# Autodesk Inventor assembly: Diamond-Box-Assembly
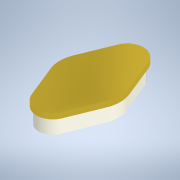
[picture p0: Inventor's stored thumbnail of the model, 180x180]
Saved by Autodesk Inventor 2022.4 (Build 264492000, 492)
## iProperties
Created: 2024-03-07
Part Number: Diamond-Box-Assembly
Document SubType Name: Assembly
Designer: t60147996
Author: t60147996
## Documents named in this file (3)
- D:\Spring 2024\Advanced CAD\Diamond Box\Diamond-Box-Assembly.iam
- D:\Spring 2024\Advanced CAD\Diamond Box\Diamond-Box.ipt
- D:\Spring 2024\Advanced CAD\Diamond Box\Diamond-Box-Lid.ipt
## Components (2 placed, 2 different names)
1. Diamond-Box:1 — Mate:1
2. Diamond-Box-Lid:1 — Mate:1
## Relationships (1: Mate 1)
- Mate:1: Diamond-Box:1 ↔ Diamond-Box-Lid:1
